# Autodesk Inventor assembly: Сборка водила
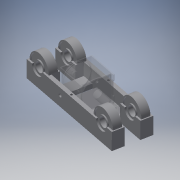
[picture p0: Inventor's stored thumbnail of the model, 180x180]
Saved by Autodesk Inventor 2017 (Build 210142000, 142)
## iProperties
Part Number: Сборка водила
Material: Типовые
Document SubType Name: Assembly
Designer: Daemon
Author: Daemon
## Documents named in this file (4)
- C:\Users\Daemon\Documents\БУ двигателем\Сборка водила.iam
- C:\Users\Daemon\Documents\БУ двигателем\Водило.ipt
- C:\Users\Daemon\Documents\БУ двигателем\Соленоид.ipt
- C:\Users\Daemon\Documents\БУ двигателем\Подшипник.ipt
## Components (6 placed, 3 different names)
1. Водило:1 — С поворотом:2, С поворотом:3, С поворотом:4, С поворотом:5, Совмещение:1, Цилиндрический:1, Цилиндрический:2, Совмещение:2
2. Соленоид:1 — Совмещение:1, Цилиндрический:1, Цилиндрический:2, Совмещение:2
3. Подшипник:1 — С поворотом:2
4. Подшипник:2 — С поворотом:3
5. Подшипник:3 — С поворотом:5
6. Подшипник:4 — С поворотом:4
## Relationships (8: RevoluteJoint 4, Mate 2, CylindricalJoint 2)
- С поворотом:2 [RevoluteJoint]: Водило:1 ↔ Подшипник:1
- С поворотом:3 [RevoluteJoint]: Водило:1 ↔ Подшипник:2
- С поворотом:4 [RevoluteJoint]: Водило:1 ↔ Подшипник:4
- С поворотом:5 [RevoluteJoint]: Водило:1 ↔ Подшипник:3
- Совмещение:1 [Mate]: Водило:1 ↔ Соленоид:1
- Цилиндрический:1 [CylindricalJoint]: Водило:1 ↔ Соленоид:1
- Цилиндрический:2 [CylindricalJoint]: Водило:1 ↔ Соленоид:1
- Совмещение:2 [Mate]: Водило:1 ↔ Соленоид:1
